# Autodesk Inventor assembly: hodoscopeHolder
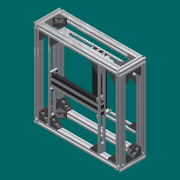
[picture p0: Inventor's stored thumbnail of the model, 180x180]
Saved by Autodesk Inventor 2016 SP1 (Build 200210100, 210)
## iProperties
Created: 2016-02-10
Part Number: hodoscopeHolder
Document SubType Name: Assembly
Designer: Sawaiz
Author: Sawaiz
## Documents named in this file (6)
- C:\Users\sawaiz\OneDrive\projects\modularHodoscope\hodoscopeBare.iam
- C:\Users\sawaiz\oneDrive\projects\modularHodoscope\fingerMount\stackBothSides.iam
- C:\Users\sawaiz\oneDrive\projects\modularHodoscope\frame\frame.iam
- C:\Users\sawaiz\oneDrive\projects\modularHodoscope\hardware\angleBracket.ipt
- C:\Users\sawaiz\oneDrive\projects\modularHodoscope\hardware\m5x10.ipt
- C:\Users\sawaiz\oneDrive\projects\modularHodoscope\hardware\m5TNut.ipt
## Components (35 placed, 5 different names)
1. frame:1 [sub-assembly] — Flush:1, Flush:2, Mate:1, Mate:2, Mate:9, Flush:3, Mate:17, Mate:33, Flush:5, Mate:34, Mate:63, Mate:64, Mate:65, Mate:66, Flush:8
2. stackBothSides:1 [sub-assembly] — Flush:2, Mate:1, Mate:10, Mate:18, Mate:25, Mate:32
3. stackBothSides:2 [sub-assembly] — Flush:1, Mate:2, Mate:59, Mate:60, Mate:61, Mate:62
4. angleBracket:1 — Mate:9, Flush:3, Mate:10, Flush:4, Symmetry:1
5. m5x10:1
6. m5x10:2
7. m5TNut:1
8. angleBracket:2 — Mate:17, Flush:4, Mate:18, Symmetry:1
9. m5x10:3
10. m5x10:4
11. m5TNut:2
12. angleBracket:3 — Mate:25, Flush:6, Mate:34
13. m5x10:5
14. m5x10:6
15. m5TNut:3
16. angleBracket:4 — Mate:32, Mate:33, Flush:5, Flush:6
17. m5x10:7
18. m5x10:8
19. m5TNut:4
20. angleBracket:5 — Mate:59, Mate:65, Flush:7, Flush:8, Flush:9, Symmetry:2
21. m5x10:9
22. m5x10:10
23. m5TNut:5
24. angleBracket:6 — Mate:60, Mate:64, Flush:9, Flush:10
25. m5x10:11
26. m5x10:12
27. m5TNut:6
28. angleBracket:7 — Mate:61, Mate:66, Flush:7, Symmetry:2
29. m5x10:13
30. m5x10:14
31. m5TNut:7
32. angleBracket:8 — Mate:62, Mate:63, Flush:10
33. m5x10:15
34. m5x10:16
35. m5TNut:8
## Relationships (86: Mate 66, Flush 10, Angle 8, Symmetry 2)
- Flush:1: frame:1 ↔ stackBothSides:2
- Flush:2: frame:1 ↔ stackBothSides:1
- Mate:1: frame:1 ↔ stackBothSides:1
- Mate:2: frame:1 ↔ stackBothSides:2
- [Mate] (2 mm): angleBracket:1 ↔ m5TNut:1
- [Angle] (0 deg): angleBracket:1 ↔ m5TNut:1
- [Mate]: angleBracket:1 ↔ m5x10:1
- [Mate]: angleBracket:1 ↔ m5x10:2
- [Mate]: angleBracket:1 ↔ m5x10:1
- [Mate]: angleBracket:1 ↔ m5x10:2
- [Mate]: m5x10:2 ↔ m5TNut:1
- Mate:9: frame:1 ↔ angleBracket:1
- Flush:3: frame:1 ↔ angleBracket:1
- Mate:10: stackBothSides:1 ↔ angleBracket:1
- [Mate] (2 mm): angleBracket:2 ↔ m5TNut:2
- [Angle] (0 deg): angleBracket:2 ↔ m5TNut:2
- [Mate]: angleBracket:2 ↔ m5x10:3
- [Mate]: angleBracket:2 ↔ m5x10:4
- [Mate]: angleBracket:2 ↔ m5x10:3
- [Mate]: angleBracket:2 ↔ m5x10:4
- [Mate]: m5x10:4 ↔ m5TNut:2
- Mate:17: frame:1 ↔ angleBracket:2
- Flush:4: angleBracket:1 ↔ angleBracket:2
- Mate:18: stackBothSides:1 ↔ angleBracket:2
- Symmetry:1: angleBracket:1 ↔ angleBracket:2
- [Mate] (2 mm): angleBracket:3 ↔ m5TNut:3
- [Angle] (0 deg): angleBracket:3 ↔ m5TNut:3
- [Mate]: angleBracket:3 ↔ m5x10:5
- [Mate]: angleBracket:3 ↔ m5x10:6
- [Mate]: angleBracket:3 ↔ m5x10:5
- [Mate]: angleBracket:3 ↔ m5x10:6
- [Mate]: m5x10:6 ↔ m5TNut:3
- Mate:25: stackBothSides:1 ↔ angleBracket:3
- [Mate] (2 mm): angleBracket:4 ↔ m5TNut:4
- [Angle] (0 deg): angleBracket:4 ↔ m5TNut:4
- [Mate]: angleBracket:4 ↔ m5x10:7
- [Mate]: angleBracket:4 ↔ m5x10:8
- [Mate]: angleBracket:4 ↔ m5x10:7
- [Mate]: angleBracket:4 ↔ m5x10:8
- [Mate]: m5x10:8 ↔ m5TNut:4
- Mate:32: stackBothSides:1 ↔ angleBracket:4
- Mate:33: frame:1 ↔ angleBracket:4
- Flush:5: frame:1 ↔ angleBracket:4
- Flush:6: angleBracket:3 ↔ angleBracket:4
- Mate:34: frame:1 ↔ angleBracket:3
- [Mate] (2 mm): angleBracket:5 ↔ m5TNut:5
- [Angle] (0 deg): angleBracket:5 ↔ m5TNut:5
- [Mate]: angleBracket:5 ↔ m5x10:9
- [Mate]: angleBracket:5 ↔ m5x10:10
- [Mate]: angleBracket:5 ↔ m5x10:9
- [Mate]: angleBracket:5 ↔ m5x10:10
- [Mate]: m5x10:10 ↔ m5TNut:5
- [Mate] (2 mm): angleBracket:6 ↔ m5TNut:6
- [Angle] (0 deg): angleBracket:6 ↔ m5TNut:6
- [Mate]: angleBracket:6 ↔ m5x10:11
- [Mate]: angleBracket:6 ↔ m5x10:12
- [Mate]: angleBracket:6 ↔ m5x10:11
- [Mate]: angleBracket:6 ↔ m5x10:12
- [Mate]: m5x10:12 ↔ m5TNut:6
- [Mate] (2 mm): angleBracket:7 ↔ m5TNut:7
- [Angle] (0 deg): angleBracket:7 ↔ m5TNut:7
- [Mate]: angleBracket:7 ↔ m5x10:13
- [Mate]: angleBracket:7 ↔ m5x10:14
- [Mate]: angleBracket:7 ↔ m5x10:13
- [Mate]: angleBracket:7 ↔ m5x10:14
- [Mate]: m5x10:14 ↔ m5TNut:7
- [Mate] (2 mm): angleBracket:8 ↔ m5TNut:8
- [Angle] (0 deg): angleBracket:8 ↔ m5TNut:8
- [Mate]: angleBracket:8 ↔ m5x10:15
- [Mate]: angleBracket:8 ↔ m5x10:16
- [Mate]: angleBracket:8 ↔ m5x10:15
- [Mate]: angleBracket:8 ↔ m5x10:16
- [Mate]: m5x10:16 ↔ m5TNut:8
- Mate:59: stackBothSides:2 ↔ angleBracket:5
- Mate:60: stackBothSides:2 ↔ angleBracket:6
- Mate:61: stackBothSides:2 ↔ angleBracket:7
- Mate:62: stackBothSides:2 ↔ angleBracket:8
- Mate:63: frame:1 ↔ angleBracket:8
- Mate:64: frame:1 ↔ angleBracket:6
- Mate:65: frame:1 ↔ angleBracket:5
- Mate:66: frame:1 ↔ angleBracket:7
- Flush:7: angleBracket:5 ↔ angleBracket:7
- Flush:8: frame:1 ↔ angleBracket:5
- Flush:9: angleBracket:5 ↔ angleBracket:6
- Flush:10: angleBracket:6 ↔ angleBracket:8
- Symmetry:2: angleBracket:5 ↔ angleBracket:7
## Named parameters: d149_d16 = 2 mm, d150_d18 = 0 deg, d151_d19 = 0 mm, d152_d20 = 0 mm, d153_d21 = 0 mm, d154_d22 = 0 mm, d155_d25 = 0 mm, d159_d16 = 2 mm, d160_d18 = 0 deg, d161_d19 = 0 mm, d162_d20 = 0 mm, d163_d21 = 0 mm, d164_d22 = 0 mm, d165_d25 = 0 mm, d167_d16 = 2 mm, d168_d18 = 0 deg, d169_d19 = 0 mm, d170_d20 = 0 mm, d171_d21 = 0 mm, d172_d22 = 0 mm, d173_d25 = 0 mm, d179_d16 = 2 mm, d180_d18 = 0 deg, d181_d19 = 0 mm, d182_d20 = 0 mm, d183_d21 = 0 mm, d184_d22 = 0 mm, d185_d25 = 0 mm, d186_d16 = 2 mm, d187_d18 = 0 deg, d188_d19 = 0 mm, d189_d20 = 0 mm, d190_d21 = 0 mm, d191_d22 = 0 mm, d192_d25 = 0 mm, d193_d16 = 2 mm, d194_d18 = 0 deg, d195_d19 = 0 mm, d196_d20 = 0 mm, d197_d21 = 0 mm, d198_d22 = 0 mm, d199_d25 = 0 mm, d200_d16 = 2 mm, d201_d18 = 0 deg, d202_d19 = 0 mm, d203_d20 = 0 mm, d204_d21 = 0 mm, d205_d22 = 0 mm, d206_d25 = 0 mm
